# Autodesk Inventor assembly: Задняя стенка
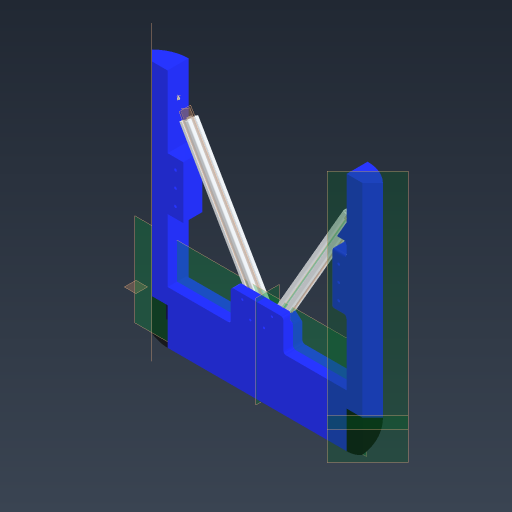
[picture p0: Inventor's stored thumbnail of the model, 512x512]
Saved by Autodesk Inventor 2023.2 (Build 272271030, 271C)
## iProperties
Created: 2025-08-20
Part Number: Задняя стенка
Document SubType Name: Assembly
Designer: Олег Коноваленко
Author: Олег Коноваленко
## Documents named in this file (7)
- D:\!Rover\Rover\Rover_construction\Задняя стенка.iam
- D:\!Rover\Rover\Rover_construction\Нижний край задней стенки.ipt
- D:\!Rover\Rover\Rover_construction\пробник.ipt
- D:\!Rover\Rover\Rover_construction\222LX-Konstruktsionnyy-profil-20kh20L.ipt
- C:\Users\I9232\Downloads\A132-Sukhar-pazovyy-M4_-paz-6\A132-Sukhar-pazovyy-M4_-paz-6.ipt
- D:\!Rover\Rover\Rover_construction\Задняя панель.ipt
- D:\!Rover\Rover\Rover_construction\Край стен.ipt
## Components (14 placed, 6 different names)
1. Нижний край задней стенки:1 — Совмещение:7, Совмещение:10, Заподлицо:8, Заподлицо:9, Заподлицо:10, Заподлицо:11, Совмещение:38, Совмещение:39, Совмещение:40, Совмещение:43, Совмещение:53, Совмещение:70, Совмещение:72, Совмещение:77, Совмещение:80, Совмещение:83
2. пробник:1 — Совмещение:7, Заподлицо:8, Совмещение:77, Совмещение:79, Совмещение:82
3. пробник:2 — Совмещение:10, Заподлицо:9, Совмещение:43, Совмещение:78, Совмещение:81
4. 222LX-Konstruktsionnyy-profil-20kh20L:1 — Заподлицо:10, Совмещение:39, Совмещение:53, Совмещение:54, Совмещение:55, Совмещение:58, Совмещение:59, Заподлицо:13, Совмещение:66, Совмещение:67
5. 222LX-Konstruktsionnyy-profil-20kh20L:2 — Заподлицо:11, Совмещение:38, Совмещение:40, Совмещение:56, Совмещение:57, Совмещение:60, Совмещение:61, Заподлицо:12, Совмещение:64, Совмещение:65
6. A132-Sukhar-pazovyy-M4_-paz-6:1 — Совмещение:54, Совмещение:59, Совмещение:63
7. A132-Sukhar-pazovyy-M4_-paz-6:2 — Совмещение:55, Совмещение:58, Совмещение:63, Заподлицо:13
8. A132-Sukhar-pazovyy-M4_-paz-6:3 — Совмещение:57, Совмещение:60, Совмещение:62, Заподлицо:12
9. A132-Sukhar-pazovyy-M4_-paz-6:4 — Совмещение:56, Совмещение:61, Совмещение:62
10. A132-Sukhar-pazovyy-M4_-paz-6:5 — Совмещение:64, Совмещение:65
11. A132-Sukhar-pazovyy-M4_-paz-6:6 — Совмещение:66, Совмещение:67
12. Задняя панель:1 — Совмещение:70, Совмещение:72, Совмещение:84
13. Край стен:1 — Совмещение:79, Совмещение:82, Совмещение:83, Совмещение:84
14. Край стен:2 — Совмещение:78, Совмещение:80, Совмещение:81
## Relationships (37: Mate 31, Flush 6)
- Совмещение:7 [Mate]: Нижний край задней стенки:1 ↔ пробник:1
- Совмещение:10 [Mate]: Нижний край задней стенки:1 ↔ пробник:2
- Заподлицо:8 [Flush]: Нижний край задней стенки:1 ↔ пробник:1
- Заподлицо:9 [Flush]: Нижний край задней стенки:1 ↔ пробник:2
- Заподлицо:10 [Flush]: Нижний край задней стенки:1 ↔ 222LX-Konstruktsionnyy-profil-20kh20L:1
- Заподлицо:11 [Flush]: Нижний край задней стенки:1 ↔ 222LX-Konstruktsionnyy-profil-20kh20L:2
- Совмещение:38 [Mate]: Нижний край задней стенки:1 ↔ 222LX-Konstruktsionnyy-profil-20kh20L:2
- Совмещение:39 [Mate]: Нижний край задней стенки:1 ↔ 222LX-Konstruktsionnyy-profil-20kh20L:1
- Совмещение:40 [Mate]: Нижний край задней стенки:1 ↔ 222LX-Konstruktsionnyy-profil-20kh20L:2
- Совмещение:43 [Mate]: Нижний край задней стенки:1 ↔ пробник:2
- Совмещение:53 [Mate]: Нижний край задней стенки:1 ↔ 222LX-Konstruktsionnyy-profil-20kh20L:1
- Совмещение:54 [Mate]: 222LX-Konstruktsionnyy-profil-20kh20L:1 ↔ A132-Sukhar-pazovyy-M4_-paz-6:1
- Совмещение:55 [Mate]: 222LX-Konstruktsionnyy-profil-20kh20L:1 ↔ A132-Sukhar-pazovyy-M4_-paz-6:2
- Совмещение:56 [Mate]: 222LX-Konstruktsionnyy-profil-20kh20L:2 ↔ A132-Sukhar-pazovyy-M4_-paz-6:4
- Совмещение:57 [Mate]: 222LX-Konstruktsionnyy-profil-20kh20L:2 ↔ A132-Sukhar-pazovyy-M4_-paz-6:3
- Совмещение:58 [Mate]: 222LX-Konstruktsionnyy-profil-20kh20L:1 ↔ A132-Sukhar-pazovyy-M4_-paz-6:2
- Совмещение:59 [Mate]: 222LX-Konstruktsionnyy-profil-20kh20L:1 ↔ A132-Sukhar-pazovyy-M4_-paz-6:1
- Совмещение:60 [Mate]: 222LX-Konstruktsionnyy-profil-20kh20L:2 ↔ A132-Sukhar-pazovyy-M4_-paz-6:3
- Совмещение:61 [Mate]: 222LX-Konstruktsionnyy-profil-20kh20L:2 ↔ A132-Sukhar-pazovyy-M4_-paz-6:4
- Совмещение:62 [Mate] (20 mm): A132-Sukhar-pazovyy-M4_-paz-6:3 ↔ A132-Sukhar-pazovyy-M4_-paz-6:4
- Совмещение:63 [Mate] (20 mm): A132-Sukhar-pazovyy-M4_-paz-6:1 ↔ A132-Sukhar-pazovyy-M4_-paz-6:2
- Заподлицо:12 [Flush]: 222LX-Konstruktsionnyy-profil-20kh20L:2 ↔ A132-Sukhar-pazovyy-M4_-paz-6:3
- Заподлицо:13 [Flush]: 222LX-Konstruktsionnyy-profil-20kh20L:1 ↔ A132-Sukhar-pazovyy-M4_-paz-6:2
- Совмещение:64 [Mate]: 222LX-Konstruktsionnyy-profil-20kh20L:2 ↔ A132-Sukhar-pazovyy-M4_-paz-6:5
- Совмещение:65 [Mate]: 222LX-Konstruktsionnyy-profil-20kh20L:2 ↔ A132-Sukhar-pazovyy-M4_-paz-6:5
- Совмещение:66 [Mate]: 222LX-Konstruktsionnyy-profil-20kh20L:1 ↔ A132-Sukhar-pazovyy-M4_-paz-6:6
- Совмещение:67 [Mate]: 222LX-Konstruktsionnyy-profil-20kh20L:1 ↔ A132-Sukhar-pazovyy-M4_-paz-6:6
- Совмещение:70 [Mate]: Нижний край задней стенки:1 ↔ Задняя панель:1
- Совмещение:72 [Mate]: Нижний край задней стенки:1 ↔ Задняя панель:1
- Совмещение:77 [Mate]: Нижний край задней стенки:1 ↔ пробник:1
- Совмещение:78 [Mate]: пробник:2 ↔ Край стен:2
- Совмещение:79 [Mate]: пробник:1 ↔ Край стен:1
- Совмещение:80 [Mate]: Нижний край задней стенки:1 ↔ Край стен:2
- Совмещение:81 [Mate]: пробник:2 ↔ Край стен:2
- Совмещение:82 [Mate]: пробник:1 ↔ Край стен:1
- Совмещение:83 [Mate]: Нижний край задней стенки:1 ↔ Край стен:1
- Совмещение:84 [Mate]: Задняя панель:1 ↔ Край стен:1
